# Autodesk Inventor assembly: Frame Test
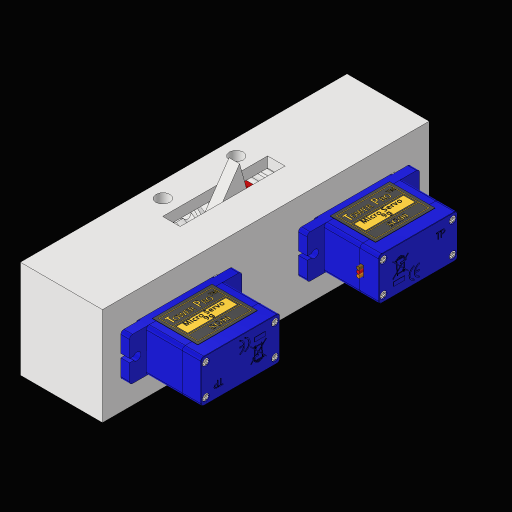
[picture p0: Inventor's stored thumbnail of the model, 512x512]
Saved by Autodesk Inventor 2023.2 (Build 272271030, 271C)
## iProperties
Created: 2023-11-06
Part Number: Frame Test
Document SubType Name: Assembly
Designer: robpl
Author: robpl
## Documents named in this file (8)
- C:\Users\robpl\OneDrive\Documents\Arduino\Onslaught\CAD\Frame Test\Frame Test.iam
- C:\Users\robpl\OneDrive\Documents\Arduino\Onslaught\CAD\Frame Test\Frame.ipt
- C:\Users\robpl\OneDrive\Documents\Arduino\Onslaught\CAD\Frame Test\SG90 - Micro Servo 9g - Tower Pro.ipt
- C:\Users\robpl\OneDrive\Documents\Arduino\Onslaught\CAD\Frame Test\Rack.ipt
- C:\Users\robpl\OneDrive\Documents\Arduino\Onslaught\CAD\Frame Test\Frame Test\Design Accelerator\Spur Gears2.iam
- C:\Users\robpl\OneDrive\Documents\Arduino\Onslaught\CAD\Frame Test\Leg.ipt
- C:\Users\robpl\OneDrive\Documents\Arduino\Onslaught\CAD\Frame Test\Frame Test\Design Accelerator\Spur Gears3.iam
- C:\Users\robpl\OneDrive\Documents\Arduino\Onslaught\CAD\Frame Test\Servo Gear.ipt
## Components (10 placed, 6 different names)
1. Frame:1 — Angle:2, Mate:12, Mate:13, Mate:14, Mate:15, Mate:16
2. SG90 - Micro Servo 9g - Tower Pro:1 — Mate:10, Mate:13, Mate:15
3. SG90 - Micro Servo 9g - Tower Pro:2 — Mate:9, Mate:11, Mate:12, Mate:14
4. Rack:1 — Flush:1, Mate:1, Flush:2, Mate:2, Mate:6, Flush:5, Angle:1
5. Spur Gears:2 [sub-assembly]
6. Leg:1 — Flush:1, Mate:1, Angle:2, Mate:16
7. Rack:2 — Flush:2, Mate:2, Mate:5, Flush:6
8. Spur Gears:3 [sub-assembly]
9. Servo Gear:1 — Mate:5, Flush:6, Mate:7, Mate:10
10. Servo Gear:2 — Mate:6, Flush:5, Mate:7, Angle:1, Mate:9, Mate:11
## Relationships (19: Mate 13, Flush 4, Angle 2)
- Flush:1: Rack:1 ↔ Leg:1
- Mate:1 (6 mm): Rack:1 ↔ Leg:1
- Flush:2: Rack:1 ↔ Rack:2
- Mate:2 (12 mm): Rack:1 ↔ Rack:2
- Mate:5 (5 mm): Rack:2 ↔ Servo Gear:1
- Mate:6 (5 mm): Rack:1 ↔ Servo Gear:2
- Flush:5: Rack:1 ↔ Servo Gear:2
- Flush:6: Rack:2 ↔ Servo Gear:1
- Mate:7: Servo Gear:1 ↔ Servo Gear:2
- Angle:1 (0 deg): Rack:1 ↔ Servo Gear:2
- Mate:9: SG90 - Micro Servo 9g - Tower Pro:2 ↔ Servo Gear:2
- Mate:10: SG90 - Micro Servo 9g - Tower Pro:1 ↔ Servo Gear:1
- Angle:2 (112.5 deg): Frame:1 ↔ Leg:1
- Mate:11: SG90 - Micro Servo 9g - Tower Pro:2 ↔ Servo Gear:2
- Mate:12: Frame:1 ↔ SG90 - Micro Servo 9g - Tower Pro:2
- Mate:13: Frame:1 ↔ SG90 - Micro Servo 9g - Tower Pro:1
- Mate:14: Frame:1 ↔ SG90 - Micro Servo 9g - Tower Pro:2
- Mate:15: Frame:1 ↔ SG90 - Micro Servo 9g - Tower Pro:1
- Mate:16 (1 mm): Frame:1 ↔ Leg:1
